# Autodesk Inventor assembly: turret_V1
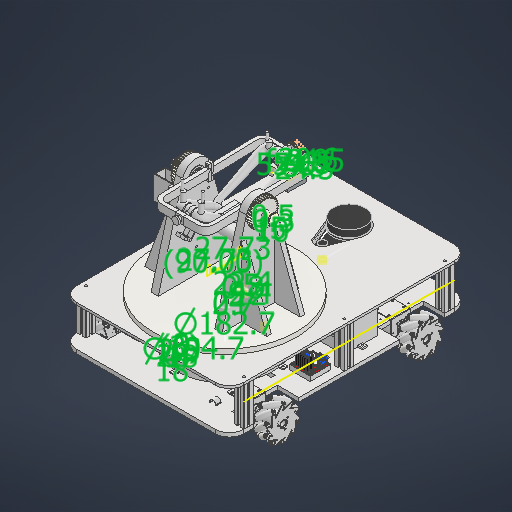
[picture p0: Inventor's stored thumbnail of the model, 512x512]
Saved by Autodesk Inventor 2026.1 (Build 301233020, 233B)
## iProperties
Created: 2025-11-28
Part Number: turret_V1
Document SubType Name: Assembly
Designer: jaewook
Author: jaewook
## Documents named in this file (41)
- C:\Users\kjh19\Documents\Inventor\project\turrte_projict_v2\turret_V1.iam
- C:\Users\kjh19\Documents\Inventor\project\turret_project\proto2\하판.ipt
- C:\Users\kjh19\Documents\Inventor\project\turret_project\final\profile.ipt
- C:\Users\kjh19\Documents\Inventor\project\turret_project\final\arduinomega.iam
- C:\Users\kjh19\Documents\Inventor\project\turret_project\final\stm32.iam
- C:\Users\kjh19\Documents\Inventor\project\turret_project\final\base_device\battery.iam
- C:\Users\kjh19\Documents\Inventor\project\turret_project\final\base_device\L298N_motor_driver.iam
- C:\Users\kjh19\Documents\Inventor\project\turret_project\proto2\motor_connector.ipt
- C:\Users\kjh19\Documents\Inventor\project\turret_project\User Library-JGB37-520-12v-319RPM.ipt
- C:\Users\kjh19\Documents\Inventor\project\turret_project\final\base_device\DC_convertor.iam
- C:\Users\kjh19\Documents\Inventor\project\turret_project\proto2\상판.ipt
- C:\Users\kjh19\Documents\Inventor\project\turret_project\proto2\example\yaw_motor_mount.iam
- C:\Users\kjh19\Documents\Inventor\project\turret_project\connector.ipt
- C:\Users\kjh19\Documents\Inventor\project\turret_project\proto2\Carrier_2.ipt
- C:\Users\kjh19\Documents\Inventor\project\turret_project\proto2\gear_support.ipt
- C:\Users\kjh19\Documents\Inventor\project\turret_project\proto2\gear_tes\디자인 액셀러레이터\스퍼 기어15.ipt
- C:\Users\kjh19\Documents\Inventor\project\turret_project\proto2\gear_tes\디자인 액셀러레이터\스퍼 기어26.ipt
- C:\Users\kjh19\Documents\Inventor\project\turret_project\proto2\gear_tes\디자인 액셀러레이터\스퍼 기어13.ipt
- C:\Users\kjh19\Documents\Inventor\project\turret_project\proto2\example\Pitch_axis.ipt
- C:\Users\kjh19\Documents\Inventor\project\turret_project\proto2\example\Pitch_axis_opp.ipt
- C:\Users\kjh19\Documents\Inventor\project\turret_project\final\custom_bearing.ipt
- C:\Users\kjh19\Documents\Inventor\project\turret_project\proto2\example\pitch_motor\디자인 액셀러레이터\스퍼 기어22.ipt
- C:\Users\kjh19\Documents\Inventor\project\turret_project\proto2\example\pitch_motor\디자인 액셀러레이터\스퍼 기어12.ipt
- C:\Users\kjh19\Documents\Inventor\project\turret_project\pitch_motor1.ipt
- C:\Users\kjh19\Documents\Inventor\project\turret_project\pitch_motor.ipt
- C:\Users\kjh19\Documents\Inventor\project\turret_project\final\roll_support_front_v2.iam
- C:\Users\kjh19\Documents\Inventor\project\turret_project\final\roll_support_left_v1.iam
- C:\Users\kjh19\Documents\Inventor\project\turret_project\final\roll_support_right.iam
- C:\Users\kjh19\Documents\Inventor\project\turret_project\final\key_v2.ipt
- C:\Users\kjh19\Documents\Inventor\project\turret_project\final\25mm_support.ipt
- C:\Users\kjh19\Documents\Inventor\project\turret_project\final\fixer.iam
- C:\Users\kjh19\Documents\Inventor\project\turret_project\final\screw_v1.ipt
- C:\Users\kjh19\Documents\Inventor\project\turret_project\final\Lidarbase.iam
- C:\Users\kjh19\Documents\Inventor\project\turret_project\final\thrust_bearing_v1.ipt
- C:\Users\kjh19\Documents\Inventor\project\turret_project\짧은 나사.ipt
- C:\Users\kjh19\Documents\Inventor\project\turret_project\Mecanum wheel 75mm L.ipt
- C:\Users\kjh19\Documents\Inventor\project\turret_project\final\roll_support_behind_v1.iam
- C:\Users\kjh19\Documents\Inventor\project\turret_project\final\base_device\battery_MIR.iam
- C:\Users\kjh19\Documents\Inventor\project\turret_project\final\pin.ipt
- C:\Users\kjh19\Documents\Inventor\project\turret_project\proto2\example\pitch_motor\디자인 액셀러레이터\스퍼 기어22_opp.ipt
- C:\Users\kjh19\Documents\Inventor\project\turret_project\final\Wire_aisle_v1.ipt
## Components (69 placed, 37 different names)
1. 하판:1 — 강체:1, 강체:2, 강체:3, 강체:4, 강체:5, 강체:6, 회전:1, 회전:2, 강체:8, 강체:9, 강체:10, 회전:3, 회전:4, 회전:5, 강체:11, 메이트:1, 메이트:2, 메이트:3, 메이트:6, 메이트:7, 메이트:9, 메이트:10, 메이트:18, 메이트:66, 메이트:67, 메이트:68, 메이트:69, 메이트:70, 메이트:71, 메이트:91, 메이트:92
2. profile:1 — 강체:1, 메이트:4
3. profile:2 — 강체:2
4. profile:3 — 강체:3, 메이트:5
5. profile:4 — 강체:4
6. profile:5 — 강체:5
7. profile:6 — 강체:6
8. arduinomega:1 [sub-assembly] — 회전:1
9. stm32:1 [sub-assembly] — 회전:2
10. battery:1 [sub-assembly]
11. L298N_motor_driver:1 [sub-assembly] — 강체:8
12. L298N_motor_driver:2 [sub-assembly] — 강체:9
13. motor_connector:2 — 강체:10, 회전:9
14. motor_connector:3 — 회전:3, 회전:8
15. motor_connector:4 — 회전:4, 회전:7
16. motor_connector:5 — 회전:5, 회전:6
17. User Library-JGB37-520-12v-319RPM:1 — 회전:6, 메이트:72, 메이트:73
18. User Library-JGB37-520-12v-319RPM:2 — 회전:7, 메이트:74, 메이트:75
19. User Library-JGB37-520-12v-319RPM:3 — 회전:8, 메이트:78, 메이트:79
20. User Library-JGB37-520-12v-319RPM:4 — 회전:9, 메이트:76, 메이트:77
21. DC_convertor:1 [sub-assembly] — 강체:11
22. DC_convertor:2 [sub-assembly] — 메이트:1, 메이트:2, 메이트:3
23. 상판:1 — 메이트:4, 메이트:5, 메이트:89, 메이트:90, 메이트:93, 메이트:94, 메이트:95
24. yaw_motor_mount:1 [sub-assembly] — 메이트:6, 메이트:7, 메이트:8, 메이트:14
25. connector:1 — 메이트:8, 메이트:11, 메이트:12, 메이트:14, 메이트:15, 메이트:24
26. Carrier_2:1 — 메이트:9, 메이트:10, 메이트:18, 메이트:19, 메이트:20, 메이트:21, 메이트:22, 메이트:23, 플러쉬:1, 메이트:104, 메이트:105
27. gear_support:2 — 메이트:11, 메이트:12, 메이트:15, 메이트:16, 메이트:17
28. 스퍼 기어1:1 — 메이트:16, 메이트:17
29. 스퍼 기어2:1 — 메이트:19, 메이트:22
30. 스퍼 기어2:2 — 메이트:20, 메이트:23, 플러쉬:2
31. 스퍼 기어2:3 — 메이트:21, 플러쉬:1
32. 스퍼 기어1:2 — 메이트:24, 플러쉬:2, 메이트:25, 메이트:26, 메이트:27, 메이트:28, 메이트:29, 메이트:30
33. Pitch_axis:1 — 메이트:25, 메이트:26, 메이트:27, 메이트:31, 메이트:32, 메이트:35, 메이트:37, 메이트:38, 메이트:44, 메이트:45
34. Pitch_axis_opp:1 — 메이트:28, 메이트:29, 메이트:30, 메이트:33, 메이트:34, 메이트:99
35. custom_bearing:1 — 메이트:31, 메이트:32, 메이트:36
36. custom_bearing:2 — 메이트:33, 메이트:34
37. 스퍼 기어2:4 — 메이트:35, 메이트:36, 메이트:59, 메이트:103
38. 스퍼 기어1:3 — 메이트:37, 메이트:38, 메이트:39, 메이트:40, 메이트:41
39. pitch_motor1:1 — 메이트:39, 메이트:40, 메이트:41
40. pitch_motor:2 — 메이트:44, 메이트:45
41. roll_support_front_v2:1 [sub-assembly] — 메이트:52, 메이트:96, 강체:12
42. roll_support_behind_v1:1 [sub-assembly] — 메이트:97, 강체:13, 메이트:98, 메이트:100, 메이트:102
43. roll_support_left_v1:1 [sub-assembly] — 메이트:49, 메이트:50, 메이트:51
44. roll_support_right:1 [sub-assembly] — 메이트:49, 메이트:50, 메이트:51, 메이트:52
45. key_v2:1 — 메이트:59
46. 25mm_support:1 — 메이트:60, 메이트:61, 메이트:66, 메이트:67
47. 25mm_support:2 — 메이트:60, 메이트:61
48. 25mm_support:3 — 메이트:62, 메이트:63, 메이트:68, 메이트:69
49. 25mm_support:4 — 메이트:62, 메이트:63
50. 25mm_support:5 — 메이트:64, 메이트:65, 메이트:70, 메이트:71
51. 25mm_support:6 — 메이트:64, 메이트:65
52. fixer:1 [sub-assembly] — 메이트:89, 메이트:90
53. screw_v1:1 — 메이트:102, 메이트:103
54. Lidarbase:1 [sub-assembly] — 메이트:93, 메이트:94, 메이트:95
55. thrust_bearing_v1:1
56. 짧은 나사:1 — 메이트:72, 메이트:73, 메이트:80, 메이트:81
57. 짧은 나사:2 — 메이트:74, 메이트:75, 메이트:82, 메이트:83
58. 짧은 나사:3 — 메이트:76, 메이트:77, 메이트:86, 메이트:87
59. 짧은 나사:4 — 메이트:78, 메이트:79, 메이트:84, 메이트:85
60. Mecanum wheel 75mm L:1 — 메이트:80, 메이트:81
61. Mecanum wheel 75mm L:2 — 메이트:82, 메이트:83
62. Mecanum wheel 75mm L:3 — 메이트:84, 메이트:85
63. Mecanum wheel 75mm L:4 — 메이트:86, 메이트:87
64. battery_MIR:1 [sub-assembly] — 메이트:91, 메이트:92
65. pin:1 — 메이트:96, 강체:12
66. pin:2 — 메이트:97, 강체:13
67. screw_v1:2 — 메이트:100, 메이트:101
68. 스퍼 기어22_opp:1 — 메이트:98, 메이트:99, 메이트:101
69. Wire_aisle_v1:1 — 메이트:104, 메이트:105
## Relationships (124: Mate 101, WeldJoint 12, RevoluteJoint 9, Flush 2)
- 강체:1 [WeldJoint]: 하판:1 ↔ profile:1
- 강체:2 [WeldJoint]: 하판:1 ↔ profile:2
- 강체:3 [WeldJoint]: 하판:1 ↔ profile:3
- 강체:4 [WeldJoint]: 하판:1 ↔ profile:4
- 강체:5 [WeldJoint]: 하판:1 ↔ profile:5
- 강체:6 [WeldJoint]: 하판:1 ↔ profile:6
- 회전:1 [RevoluteJoint]: 하판:1 ↔ arduinomega:1
- 회전:2 [RevoluteJoint]: 하판:1 ↔ stm32:1
- 강체:8 [WeldJoint]: 하판:1 ↔ L298N_motor_driver:1
- 강체:9 [WeldJoint]: 하판:1 ↔ L298N_motor_driver:2
- 강체:10 [WeldJoint]: 하판:1 ↔ motor_connector:2
- 회전:3 [RevoluteJoint]: 하판:1 ↔ motor_connector:3
- 회전:4 [RevoluteJoint]: 하판:1 ↔ motor_connector:4
- 회전:5 [RevoluteJoint]: 하판:1 ↔ motor_connector:5
- 회전:6 [RevoluteJoint]: motor_connector:5 ↔ User Library-JGB37-520-12v-319RPM:1
- 회전:7 [RevoluteJoint]: motor_connector:4 ↔ User Library-JGB37-520-12v-319RPM:2
- 회전:8 [RevoluteJoint]: motor_connector:3 ↔ User Library-JGB37-520-12v-319RPM:3
- 회전:9 [RevoluteJoint]: motor_connector:2 ↔ User Library-JGB37-520-12v-319RPM:4
- 강체:11 [WeldJoint]: 하판:1 ↔ DC_convertor:1
- 메이트:1 [Mate]: 하판:1 ↔ DC_convertor:2
- 메이트:2 [Mate]: 하판:1 ↔ DC_convertor:2
- 메이트:3 [Mate]: 하판:1 ↔ DC_convertor:2
- 메이트:4 [Mate]: profile:1 ↔ 상판:1
- 메이트:5 [Mate]: profile:3 ↔ 상판:1
- 메이트:6 [Mate]: 하판:1 ↔ yaw_motor_mount:1
- 메이트:7 [Mate]: 하판:1 ↔ yaw_motor_mount:1
- 메이트:8 [Mate]: yaw_motor_mount:1 ↔ connector:1
- 메이트:9 [Mate]: 하판:1 ↔ Carrier_2:1
- 메이트:10 [Mate]: 하판:1 ↔ Carrier_2:1
- 메이트:11 [Mate]: connector:1 ↔ gear_support:2
- 메이트:12 [Mate]: connector:1 ↔ gear_support:2
- 메이트:14 [Mate]: yaw_motor_mount:1 ↔ connector:1
- 메이트:15 [Mate]: connector:1 ↔ gear_support:2
- 메이트:16 [Mate]: gear_support:2 ↔ 스퍼 기어1:1
- 메이트:17 [Mate]: gear_support:2 ↔ 스퍼 기어1:1
- 메이트:18 [Mate]: 하판:1 ↔ Carrier_2:1
- 메이트:19 [Mate]: Carrier_2:1 ↔ 스퍼 기어2:1
- 메이트:20 [Mate]: Carrier_2:1 ↔ 스퍼 기어2:2
- 메이트:21 [Mate]: Carrier_2:1 ↔ 스퍼 기어2:3
- 메이트:22 [Mate]: Carrier_2:1 ↔ 스퍼 기어2:1
- 메이트:23 [Mate]: Carrier_2:1 ↔ 스퍼 기어2:2
- 플러쉬:1 [Flush]: Carrier_2:1 ↔ 스퍼 기어2:3
- 메이트:24 [Mate]: connector:1 ↔ 스퍼 기어1:2
- 플러쉬:2 [Flush]: 스퍼 기어2:2 ↔ 스퍼 기어1:2
- 메이트:25 [Mate] (0.25 mm): 스퍼 기어1:2 ↔ Pitch_axis:1
- 메이트:26 [Mate]: 스퍼 기어1:2 ↔ Pitch_axis:1
- 메이트:27 [Mate]: 스퍼 기어1:2 ↔ Pitch_axis:1
- 메이트:28 [Mate] (0.25 mm): 스퍼 기어1:2 ↔ Pitch_axis_opp:1
- 메이트:29 [Mate]: 스퍼 기어1:2 ↔ Pitch_axis_opp:1
- 메이트:30 [Mate]: 스퍼 기어1:2 ↔ Pitch_axis_opp:1
- 메이트:31 [Mate]: Pitch_axis:1 ↔ custom_bearing:1
- 메이트:32 [Mate]: Pitch_axis:1 ↔ custom_bearing:1
- 메이트:33 [Mate]: Pitch_axis_opp:1 ↔ custom_bearing:2
- 메이트:34 [Mate]: Pitch_axis_opp:1 ↔ custom_bearing:2
- 메이트:35 [Mate]: Pitch_axis:1 ↔ 스퍼 기어2:4
- 메이트:36 [Mate]: custom_bearing:1 ↔ 스퍼 기어2:4
- 메이트:37 [Mate]: Pitch_axis:1 ↔ 스퍼 기어1:3
- 메이트:38 [Mate]: Pitch_axis:1 ↔ 스퍼 기어1:3
- 메이트:39 [Mate]: 스퍼 기어1:3 ↔ pitch_motor1:1
- 메이트:40 [Mate]: 스퍼 기어1:3 ↔ pitch_motor1:1
- 메이트:41 [Mate]: 스퍼 기어1:3 ↔ pitch_motor1:1
- 메이트:44 [Mate]: Pitch_axis:1 ↔ pitch_motor:2
- 메이트:45 [Mate]: Pitch_axis:1 ↔ pitch_motor:2
- [Mate]: roll_support_front_v2:1 ↔ roll_support_behind_v1:1
- [Mate]: roll_support_front_v2:1 ↔ roll_support_behind_v1:1
- [Mate]: roll_support_front_v2:1 ↔ roll_support_behind_v1:1
- 메이트:49 [Mate]: roll_support_left_v1:1 ↔ roll_support_right:1
- 메이트:50 [Mate]: roll_support_left_v1:1 ↔ roll_support_right:1
- 메이트:51 [Mate]: roll_support_left_v1:1 ↔ roll_support_right:1
- 메이트:52 [Mate]: roll_support_front_v2:1 ↔ roll_support_right:1
- [Mate]: roll_support_behind_v1:1 ↔ roll_support_right:1
- [Mate]: custom_bearing:1 ↔ roll_support_behind_v1:1
- [Mate]: roll_support_behind_v1:1 ↔ key_v2:1
- [Mate]: roll_support_behind_v1:1 ↔ key_v2:1
- [Mate]: roll_support_behind_v1:1 ↔ key_v2:1
- [Mate]: Pitch_axis:1 ↔ roll_support_behind_v1:1
- 메이트:59 [Mate]: 스퍼 기어2:4 ↔ key_v2:1
- 메이트:60 [Mate]: 25mm_support:1 ↔ 25mm_support:2
- 메이트:61 [Mate]: 25mm_support:1 ↔ 25mm_support:2
- 메이트:62 [Mate]: 25mm_support:3 ↔ 25mm_support:4
- 메이트:63 [Mate]: 25mm_support:3 ↔ 25mm_support:4
- 메이트:64 [Mate]: 25mm_support:5 ↔ 25mm_support:6
- 메이트:65 [Mate]: 25mm_support:5 ↔ 25mm_support:6
- 메이트:66 [Mate]: 하판:1 ↔ 25mm_support:1
- 메이트:67 [Mate]: 하판:1 ↔ 25mm_support:1
- 메이트:68 [Mate]: 하판:1 ↔ 25mm_support:3
- 메이트:69 [Mate]: 하판:1 ↔ 25mm_support:3
- 메이트:70 [Mate]: 하판:1 ↔ 25mm_support:5
- 메이트:71 [Mate]: 하판:1 ↔ 25mm_support:5
- 메이트:72 [Mate]: User Library-JGB37-520-12v-319RPM:1 ↔ 짧은 나사:1
- 메이트:73 [Mate]: User Library-JGB37-520-12v-319RPM:1 ↔ 짧은 나사:1
- 메이트:74 [Mate]: User Library-JGB37-520-12v-319RPM:2 ↔ 짧은 나사:2
- 메이트:75 [Mate]: User Library-JGB37-520-12v-319RPM:2 ↔ 짧은 나사:2
- 메이트:76 [Mate]: User Library-JGB37-520-12v-319RPM:4 ↔ 짧은 나사:3
- 메이트:77 [Mate]: User Library-JGB37-520-12v-319RPM:4 ↔ 짧은 나사:3
- 메이트:78 [Mate]: User Library-JGB37-520-12v-319RPM:3 ↔ 짧은 나사:4
- 메이트:79 [Mate]: User Library-JGB37-520-12v-319RPM:3 ↔ 짧은 나사:4
- 메이트:80 [Mate]: 짧은 나사:1 ↔ Mecanum wheel 75mm L:1
- 메이트:81 [Mate]: 짧은 나사:1 ↔ Mecanum wheel 75mm L:1
- 메이트:82 [Mate]: 짧은 나사:2 ↔ Mecanum wheel 75mm L:2
- 메이트:83 [Mate]: 짧은 나사:2 ↔ Mecanum wheel 75mm L:2
- 메이트:84 [Mate]: 짧은 나사:4 ↔ Mecanum wheel 75mm L:3
- 메이트:85 [Mate]: 짧은 나사:4 ↔ Mecanum wheel 75mm L:3
- 메이트:86 [Mate]: 짧은 나사:3 ↔ Mecanum wheel 75mm L:4
- 메이트:87 [Mate]: 짧은 나사:3 ↔ Mecanum wheel 75mm L:4
- 메이트:89 [Mate]: 상판:1 ↔ fixer:1
- 메이트:90 [Mate]: 상판:1 ↔ fixer:1
- 메이트:91 [Mate]: 하판:1 ↔ battery_MIR:1
- 메이트:92 [Mate]: 하판:1 ↔ battery_MIR:1
- 메이트:93 [Mate]: 상판:1 ↔ Lidarbase:1
- 메이트:94 [Mate]: 상판:1 ↔ Lidarbase:1
- 메이트:95 [Mate]: 상판:1 ↔ Lidarbase:1
- 메이트:96 [Mate]: roll_support_front_v2:1 ↔ pin:1
- 강체:12 [WeldJoint]: roll_support_front_v2:1 ↔ pin:1
- 메이트:97 [Mate]: roll_support_behind_v1:1 ↔ pin:2
- 강체:13 [WeldJoint]: roll_support_behind_v1:1 ↔ pin:2
- 메이트:98 [Mate]: roll_support_behind_v1:1 ↔ 스퍼 기어22_opp:1
- 메이트:99 [Mate]: Pitch_axis_opp:1 ↔ 스퍼 기어22_opp:1
- 메이트:100 [Mate]: roll_support_behind_v1:1 ↔ screw_v1:2
- 메이트:101 [Mate]: screw_v1:2 ↔ 스퍼 기어22_opp:1
- 메이트:102 [Mate]: roll_support_behind_v1:1 ↔ screw_v1:1
- 메이트:103 [Mate]: 스퍼 기어2:4 ↔ screw_v1:1
- 메이트:104 [Mate]: Carrier_2:1 ↔ Wire_aisle_v1:1
- 메이트:105 [Mate]: Carrier_2:1 ↔ Wire_aisle_v1:1
